# Autodesk Inventor assembly: postStandSupport
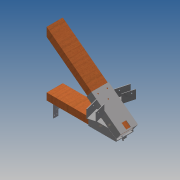
[picture p0: Inventor's stored thumbnail of the model, 180x180]
Saved by Autodesk Inventor 2014 SP1 (Build 180222100, 222)
## iProperties
Created: 2014-08-29
Part Number: postStandSupport
Document SubType Name: Assembly
Designer: Dave
Author: Dave
## Documents named in this file (5)
- C:\Users\Dave\Desktop\hera-cad\support\postStandSupport.iam
- C:\Users\Dave\Desktop\hera-cad\support\postStandHoriz.ipt
- C:\Users\Dave\Desktop\hera-cad\support\endAssembly.iam
- C:\Users\Dave\Desktop\hera-cad\support\postStand37.ipt
- C:\Users\Dave\Desktop\hera-cad\smallParts\angleBracket.ipt
## Components (4 placed, 4 different names)
1. postStandHoriz:1 — Mate:1, Mate:2, Mate:3, Mate:7, Flush:1
2. endAssembly:1 [sub-assembly] — Mate:1, Mate:2, Mate:3, Mate:4, Mate:5, Mate:6
3. postStand37:1 — Mate:4, Mate:5, Mate:6
4. angleBracket:1 — Mate:7, Flush:1
## Relationships (8: Mate 7, Flush 1)
- Mate:1: postStandHoriz:1 ↔ endAssembly:1
- Mate:2: postStandHoriz:1 ↔ endAssembly:1
- Mate:3: postStandHoriz:1 ↔ endAssembly:1
- Mate:4: endAssembly:1 ↔ postStand37:1
- Mate:5: endAssembly:1 ↔ postStand37:1
- Mate:6: endAssembly:1 ↔ postStand37:1
- Mate:7: postStandHoriz:1 ↔ angleBracket:1
- Flush:1: postStandHoriz:1 ↔ angleBracket:1
